# Autodesk Inventor assembly: !Crossbrace
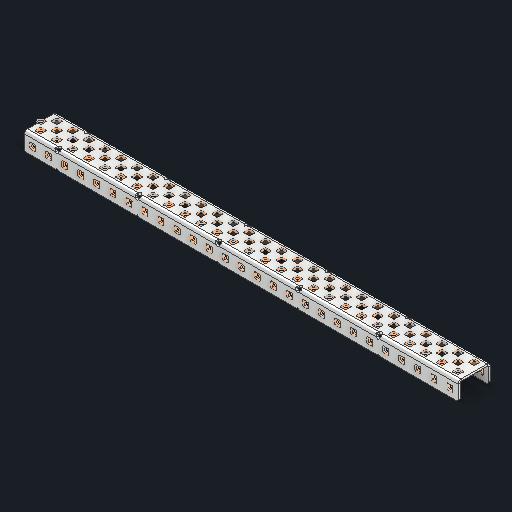
[picture p0: Inventor's stored thumbnail of the model, 512x512]
Saved by Autodesk Inventor 2025.1 (Build 291241000, 241)
## iProperties
Created: 2024-12-18
Part Number: !Crossbrace
Document SubType Name: Assembly
Designer: avere
Author: avere
## Documents named in this file (2)
- C:\Users\avere\VEX\High Stakes\CAD\V4\Chassis\Crossbrace\!Crossbrace.iam
- C:\Users\avere\VEX\High Stakes\CAD\ROBOPROS-CAD-Inventor\Structure\C Channel\Aluminum 1x2x1\Alu C 1x2x1x27.ipt
## Components (1 placed, 1 different names)
1. Alu C 1x2x1x27:1 — Mate:1, Flush:1, Flush:2
## Relationships (3: Flush 2, Mate 1)
- Mate:1 (88.9 mm): Alu C 1x2x1x27:1
- Flush:1 (-171.45 mm): Alu C 1x2x1x27:1
- Flush:2 (-17.4625 mm): Alu C 1x2x1x27:1
